# Autodesk Inventor assembly: napinacz_zlozenie_final
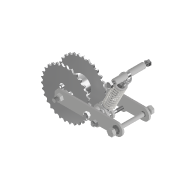
[picture p0: Inventor's stored thumbnail of the model, 180x180]
Saved by Autodesk Inventor 2020.3 (Build 243373000, 373)
## iProperties
Created: 2021-11-03
Part Number: napinacz_zlozenie_final
Document SubType Name: Assembly
Designer: patry
Author: patry
## Documents named in this file (18)
- C:\Users\patry\Desktop\Semestr 7\Inzynierka\Projekt inventor\Ariadna_inzynierka\Workspaces\Obszar roboczy\Obszar roboczy\Naped\Zawieszenie_v3\napinacz_zlozenie_final.iam
- C:\Users\patry\Desktop\Semestr 7\Inzynierka\Projekt inventor\Ariadna_inzynierka\Workspaces\Obszar roboczy\Obszar roboczy\Naped\Kola\kolo_przednie.iam
- C:\Users\patry\Desktop\Semestr 7\Inzynierka\Projekt inventor\Ariadna_inzynierka\Workspaces\Obszar roboczy\Obszar roboczy\Naped\Zawieszenie_v3\ramie_napinacza.ipt
- C:\Users\patry\Desktop\Semestr 7\Inzynierka\Projekt inventor\Ariadna_inzynierka\Workspaces\Obszar roboczy\Obszar roboczy\Naped\Sruby\M5_nut_5mm.ipt
- C:\Users\patry\Desktop\Semestr 7\Inzynierka\Projekt inventor\Ariadna_inzynierka\Workspaces\Obszar roboczy\Obszar roboczy\Naped\Sruby\M5_70_shaft.ipt
- C:\Users\patry\Desktop\Semestr 7\Inzynierka\Projekt inventor\Ariadna_inzynierka\Workspaces\Obszar roboczy\Obszar roboczy\Naped\Sruby\M3_16_shaft.ipt
- C:\Users\patry\Desktop\Semestr 7\Inzynierka\Projekt inventor\Ariadna_inzynierka\Workspaces\Obszar roboczy\Obszar roboczy\Naped\Sruby\M3_nut_2,5mm.ipt
- C:\Users\patry\Desktop\Semestr 7\Inzynierka\Projekt inventor\Ariadna_inzynierka\Workspaces\Obszar roboczy\Obszar roboczy\Naped\Zawieszenie_v3\wspornik_amortyzatora.ipt
- C:\Users\patry\Desktop\Semestr 7\Inzynierka\Projekt inventor\Ariadna_inzynierka\Workspaces\Obszar roboczy\Obszar roboczy\Naped\Sruby\tuleja_M5_M9_20.ipt
- C:\Users\patry\Desktop\Semestr 7\Inzynierka\Projekt inventor\Ariadna_inzynierka\Workspaces\Obszar roboczy\Obszar roboczy\Naped\Sruby\tuleja_M5_M9_25.ipt
- C:\Users\patry\Desktop\Semestr 7\Inzynierka\Projekt inventor\Ariadna_inzynierka\Workspaces\Obszar roboczy\Obszar roboczy\Naped\Sruby\M5_60_shaft.ipt
- C:\Users\patry\Desktop\Semestr 7\Inzynierka\Projekt inventor\Ariadna_inzynierka\Workspaces\Obszar roboczy\Obszar roboczy\Naped\Zawieszenie_v3\tuleja_TUF106040.ipt
- C:\Users\patry\Desktop\Semestr 7\Inzynierka\Projekt inventor\Ariadna_inzynierka\Workspaces\Obszar roboczy\Obszar roboczy\Naped\Sruby\M6_70_shaft.ipt
- C:\Users\patry\Desktop\Semestr 7\Inzynierka\Projekt inventor\Ariadna_inzynierka\Workspaces\Obszar roboczy\Obszar roboczy\Naped\Sruby\M6_nut_5mm.ipt
- C:\Users\patry\Desktop\Semestr 7\Inzynierka\Projekt inventor\Ariadna_inzynierka\Workspaces\Obszar roboczy\Obszar roboczy\Naped\Sruby\tuleja_M5_M9_13.ipt
- C:\Users\patry\Desktop\Semestr 7\Inzynierka\Projekt inventor\Ariadna_inzynierka\Workspaces\Obszar roboczy\Obszar roboczy\Naped\Sruby\tuleja_M5_M9_18.ipt
- C:\Users\patry\Desktop\Semestr 7\Inzynierka\Projekt inventor\Ariadna_inzynierka\Workspaces\Obszar roboczy\Obszar roboczy\Naped\Sruby\tuleja_M6_M10_8.ipt
- C:\Users\patry\Desktop\Semestr 7\Inzynierka\Projekt inventor\Ariadna_inzynierka\Workspaces\Obszar roboczy\Obszar roboczy\Naped\Amortyzator\elemenet_sprężysty.iam
## Components (32 placed, 18 different names)
1. kolo_przednie:1 [sub-assembly] — Zestawiające:57, Zestawiające:58
2. ramie_napinacza:1 — Zestawiające:49, Zestawiające:50, Zestawiające:51, Zestawiające:52, Zestawiające:53, Zestawiające:57, Zestawiające:58, Zestawiające:59, Równoległe:4, Zestawiające:60, Równoległe:5, Zestawiające:64, Zestawiające:70, Zestawiające:74, Zestawiające:75, Równoległe:7, Zestawiające:77, Zestawiające:81, Kątowe:1, Kątowe:2, Równoległe:10, Kątowe:3
3. M5_nakretka_5mm:1 — Równoległe:6
4. M5_70_shaft:1 — Zestawiające:84, Równoległe:9
5. M5_nut_5mm:2 — Równoległe:9
6. M5_nut_5mm:3 — Zestawiające:69, Zestawiające:70
7. M5_nut_5mm:4 — Zestawiające:61, Zestawiające:64
8. M5_nut_5mm:5 — Zestawiające:65, Zestawiające:66
9. M5_nut_5mm:6 — Zestawiające:67, Zestawiające:68
10. tuleja_M5_M9_20:1 — Zestawiające:85
11. tuleja_M5_M9_25:1 — Zestawiające:99
12. ramie_napinacza:2 — Zestawiające:49, Zestawiające:50, Zestawiające:51, Zestawiające:54, Zestawiające:55, Równoległe:3, Zestawiające:66, Zestawiające:68, Zestawiające:79, Zestawiające:83, Równoległe:10, Kątowe:4
13. M5_60_shaft:1 — Zestawiające:59, Równoległe:4, Zestawiające:61, Zestawiające:65, Zestawiające:71, Zestawiające:73, Zestawiające:94
14. M5_60_shaft:2 — Zestawiające:60, Równoległe:5, Zestawiające:67, Zestawiające:69, Zestawiające:95
15. tuleja_TUF106040:1 — Zestawiające:52, Zestawiające:53, Zestawiające:56
16. tuleja_TUF106040:2 — Zestawiające:54, Zestawiające:55
17. M6_70_shaft:1 — Równoległe:3
18. M6_nut_5mm:1 — Zestawiające:56
19. M6_nut_5mm:2 — Równoległe:6
20. tuleja_M5_M9_13:1 — Zestawiające:73, Zestawiające:74, Zestawiające:96
21. tuleja_M5_M9_18:1 — Zestawiające:71
22. M6_70_shaft:2 — Zestawiające:75, Równoległe:7, Zestawiające:76, Zestawiające:78, Zestawiające:80, Zestawiające:82
23. M6_nut_5mm:3 — Zestawiające:76, Zestawiające:77
24. M6_nut_5mm:4 — Zestawiające:78, Zestawiające:79
25. tuleja_M6_M10_8:1 — Zestawiające:80, Zestawiające:81
26. tuleja_M6_M10_8:2 — Zestawiające:82, Zestawiające:83
27. elemenet_sprężysty:1 [sub-assembly] — Zestawiające:84, Zestawiające:85, Zestawiające:97, Zestawiające:98, Kątowe:2, Zestawiające:99
28. M3_16_shaft:2 — Zestawiające:97
29. M3_nut_2,5mm:3
30. M3_nut_2,5mm:4
31. mocowanie_sprężyny:1 — Zestawiające:94, Zestawiające:95, Zestawiające:96, Zestawiające:98
32. mocowanie_sprężyny:2
## Relationships (69: Mate 57, Flush 8, Angle 4)
- [Mate]: M5_nakretka_5mm:1 ↔ M5_70_shaft:1
- [Mate]: M5_70_shaft:1 ↔ M5_nut_5mm:2
- [Mate] (60 mm): M5_nakretka_5mm:1 ↔ M5_nut_5mm:2
- [Mate]: M5_70_shaft:1 ↔ tuleja_M5_M9_20:1
- [Mate]: M5_70_shaft:1 ↔ tuleja_M5_M9_25:1
- [Mate]: M6_70_shaft:1 ↔ M6_nut_5mm:1
- [Mate]: M6_70_shaft:1 ↔ M6_nut_5mm:2
- [Mate] (60 mm): M6_nut_5mm:1 ↔ M6_nut_5mm:2
- [Mate]: tuleja_TUF106040:1 ↔ M6_70_shaft:1
- Zestawiające:49 [Mate]: ramie_napinacza:1 ↔ ramie_napinacza:2
- Zestawiające:50 [Mate]: ramie_napinacza:1 ↔ ramie_napinacza:2
- Zestawiające:51 [Mate] (42 mm): ramie_napinacza:1 ↔ ramie_napinacza:2
- Zestawiające:52 [Mate]: ramie_napinacza:1 ↔ tuleja_TUF106040:1
- Zestawiające:53 [Mate]: ramie_napinacza:1 ↔ tuleja_TUF106040:1
- Zestawiające:54 [Mate]: ramie_napinacza:2 ↔ tuleja_TUF106040:2
- Zestawiające:55 [Mate]: ramie_napinacza:2 ↔ tuleja_TUF106040:2
- Zestawiające:56 [Mate] (5 mm): tuleja_TUF106040:1 ↔ M6_nut_5mm:1
- Równoległe:3 [Flush] (-11 mm): ramie_napinacza:2 ↔ M6_70_shaft:1
- Zestawiające:57 [Mate] (5.5 mm): kolo_przednie:1 ↔ ramie_napinacza:1
- Zestawiające:58 [Mate]: kolo_przednie:1 ↔ ramie_napinacza:1
- Zestawiające:59 [Mate]: ramie_napinacza:1 ↔ M5_60_shaft:1
- Równoległe:4 [Flush] (6 mm): ramie_napinacza:1 ↔ M5_60_shaft:1
- Zestawiające:60 [Mate]: ramie_napinacza:1 ↔ M5_60_shaft:2
- Równoległe:5 [Flush] (6 mm): ramie_napinacza:1 ↔ M5_60_shaft:2
- Zestawiające:61 [Mate]: M5_nut_5mm:4 ↔ M5_60_shaft:1
- Zestawiające:64 [Mate]: ramie_napinacza:1 ↔ M5_nut_5mm:4
- Zestawiające:65 [Mate]: M5_nut_5mm:5 ↔ M5_60_shaft:1
- Zestawiające:66 [Mate]: M5_nut_5mm:5 ↔ ramie_napinacza:2
- Zestawiające:67 [Mate]: M5_nut_5mm:6 ↔ M5_60_shaft:2
- Zestawiające:68 [Mate]: M5_nut_5mm:6 ↔ ramie_napinacza:2
- Zestawiające:69 [Mate]: M5_nut_5mm:3 ↔ M5_60_shaft:2
- Zestawiające:70 [Mate]: ramie_napinacza:1 ↔ M5_nut_5mm:3
- Równoległe:6 [Flush]: M5_nakretka_5mm:1 ↔ M6_nut_5mm:2
- Zestawiające:71 [Mate]: M5_60_shaft:1 ↔ tuleja_M5_M9_18:1
- Zestawiające:73 [Mate]: M5_60_shaft:1 ↔ tuleja_M5_M9_13:1
- Zestawiające:74 [Mate]: ramie_napinacza:1 ↔ tuleja_M5_M9_13:1
- Zestawiające:75 [Mate]: ramie_napinacza:1 ↔ M6_70_shaft:2
- Równoległe:7 [Flush] (-11 mm): ramie_napinacza:1 ↔ M6_70_shaft:2
- Zestawiające:76 [Mate]: M6_70_shaft:2 ↔ M6_nut_5mm:3
- Zestawiające:77 [Mate]: ramie_napinacza:1 ↔ M6_nut_5mm:3
- Zestawiające:78 [Mate]: M6_70_shaft:2 ↔ M6_nut_5mm:4
- Zestawiające:79 [Mate]: ramie_napinacza:2 ↔ M6_nut_5mm:4
- Zestawiające:80 [Mate]: M6_70_shaft:2 ↔ tuleja_M6_M10_8:1
- Zestawiające:81 [Mate]: ramie_napinacza:1 ↔ tuleja_M6_M10_8:1
- Zestawiające:82 [Mate]: M6_70_shaft:2 ↔ tuleja_M6_M10_8:2
- Zestawiające:83 [Mate]: ramie_napinacza:2 ↔ tuleja_M6_M10_8:2
- Zestawiające:84 [Mate]: M5_70_shaft:1 ↔ elemenet_sprężysty:1
- Zestawiające:85 [Mate]: tuleja_M5_M9_20:1 ↔ elemenet_sprężysty:1
- [Mate]: mocowanie_sprężyny:1 ↔ mocowanie_sprężyny:2
- [Mate]: mocowanie_sprężyny:1 ↔ mocowanie_sprężyny:2
- [Mate] (5 mm): mocowanie_sprężyny:1 ↔ mocowanie_sprężyny:2
- [Mate]: M3_16_shaft:2 ↔ mocowanie_sprężyny:2
- [Flush] (-2.5 mm): M3_16_shaft:2 ↔ mocowanie_sprężyny:1
- [Mate]: M3_16_shaft:2 ↔ M3_nut_2,5mm:3
- [Mate]: M3_nut_2,5mm:3 ↔ mocowanie_sprężyny:1
- [Mate]: M3_16_shaft:2 ↔ M3_nut_2,5mm:4
- [Mate]: M3_nut_2,5mm:4 ↔ mocowanie_sprężyny:2
- Zestawiające:94 [Mate]: M5_60_shaft:1 ↔ mocowanie_sprężyny:1
- Zestawiające:95 [Mate]: M5_60_shaft:2 ↔ mocowanie_sprężyny:1
- Zestawiające:96 [Mate]: tuleja_M5_M9_13:1 ↔ mocowanie_sprężyny:1
- Zestawiające:97 [Mate]: elemenet_sprężysty:1 ↔ M3_16_shaft:2
- Kątowe:1 [Angle] (0 deg): ramie_napinacza:1
- Zestawiające:98 [Mate]: elemenet_sprężysty:1 ↔ mocowanie_sprężyny:1
- Równoległe:9 [Flush]: M5_70_shaft:1 ↔ M5_nut_5mm:2
- Kątowe:2 [Angle] (152.25 deg): ramie_napinacza:1 ↔ elemenet_sprężysty:1
- Równoległe:10 [Flush]: ramie_napinacza:1 ↔ ramie_napinacza:2
- Kątowe:3 [Angle] (90 deg): ramie_napinacza:1
- Zestawiające:99 [Mate]: tuleja_M5_M9_25:1 ↔ elemenet_sprężysty:1
- Kątowe:4 [Angle] (0 deg): ramie_napinacza:2
## Named parameters: d102_d120 = 0 mm, d103_d121 = 0 mm, d104_d122 = 5 mm, d105_d123 = 0 mm, d106_d124 = -2.5 mm, d107_d125 = 0 mm, d108_d126 = 0 mm, d109_d127 = 0 mm, d113_d128 = 0 mm
